# Autodesk Inventor assembly: Mini Power Module (REV-11-1956)
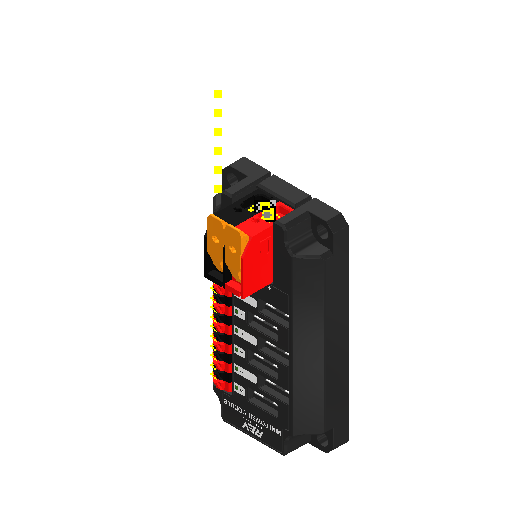
[picture p0: Inventor's stored thumbnail of the model, 512x512]
Saved by Autodesk Inventor 2023 (Build 270158000, 158)
## iProperties
Created: 2023-04-23
Part Number: Mini Power Module (REV-11-1956)
Description: STEP AP242
Document SubType Name: Assembly
Designer: adamarnold
Preprocessor: ST-DEVELOPER v18.102
Title: 64447f9ab2ee3a2914539952
## Documents named in this file (91)
- J:\My Drive\1939\2_Design\2023-2024\Parts\Electronics\Power Delivery\Mini Power Module (REV-11-1956).iam
- J:\My Drive\1939\2_Design\2023-2024\Parts\Electronics\MPM Parts\REV-11-1956.ipt
- J:\My Drive\1939\2_Design\2023-2024\Parts\Electronics\MPM Parts\REV-11-1956_1.ipt
- J:\My Drive\1939\2_Design\2023-2024\Parts\Electronics\MPM Parts\REV-11-1956_2.ipt
- J:\My Drive\1939\2_Design\2023-2024\Parts\Electronics\MPM Parts\REV-11-1956_3.ipt
- J:\My Drive\1939\2_Design\2023-2024\Parts\Electronics\MPM Parts\REV-11-1956_4.ipt
- J:\My Drive\1939\2_Design\2023-2024\Parts\Electronics\MPM Parts\REV-11-1956_5.ipt
- J:\My Drive\1939\2_Design\2023-2024\Parts\Electronics\MPM Parts\REV-11-1956_7.ipt
- J:\My Drive\1939\2_Design\2023-2024\Parts\Electronics\MPM Parts\REV-11-1956_8.ipt
- J:\My Drive\1939\2_Design\2023-2024\Parts\Electronics\MPM Parts\REV-11-1956_9.ipt
- J:\My Drive\1939\2_Design\2023-2024\Parts\Electronics\MPM Parts\REV-11-1956_10.ipt
- J:\My Drive\1939\2_Design\2023-2024\Parts\Electronics\MPM Parts\REV-11-1956_11.ipt
- J:\My Drive\1939\2_Design\2023-2024\Parts\Electronics\MPM Parts\REV-11-1956_12.ipt
- J:\My Drive\1939\2_Design\2023-2024\Parts\Electronics\MPM Parts\REV-11-1956_14.ipt
- J:\My Drive\1939\2_Design\2023-2024\Parts\Electronics\MPM Parts\REV-11-1956_15.ipt
- J:\My Drive\1939\2_Design\2023-2024\Parts\Electronics\MPM Parts\REV-11-1956_16.ipt
- J:\My Drive\1939\2_Design\2023-2024\Parts\Electronics\MPM Parts\REV-11-1956_17.ipt
- J:\My Drive\1939\2_Design\2023-2024\Parts\Electronics\MPM Parts\REV-11-1956_18.ipt
- J:\My Drive\1939\2_Design\2023-2024\Parts\Electronics\MPM Parts\REV-11-1956_19.ipt
- J:\My Drive\1939\2_Design\2023-2024\Parts\Electronics\MPM Parts\REV-11-1956_20.ipt
- J:\My Drive\1939\2_Design\2023-2024\Parts\Electronics\MPM Parts\REV-11-1956_22.ipt
- J:\My Drive\1939\2_Design\2023-2024\Parts\Electronics\MPM Parts\REV-11-1956_23.ipt
- J:\My Drive\1939\2_Design\2023-2024\Parts\Electronics\MPM Parts\REV-11-1956_24.ipt
- J:\My Drive\1939\2_Design\2023-2024\Parts\Electronics\MPM Parts\REV-11-1956_25.ipt
- J:\My Drive\1939\2_Design\2023-2024\Parts\Electronics\MPM Parts\REV-11-1956_26.ipt
- J:\My Drive\1939\2_Design\2023-2024\Parts\Electronics\MPM Parts\REV-11-1956_27.ipt
- J:\My Drive\1939\2_Design\2023-2024\Parts\Electronics\MPM Parts\REV-11-1956_29.ipt
- J:\My Drive\1939\2_Design\2023-2024\Parts\Electronics\MPM Parts\REV-11-1956_30.ipt
- J:\My Drive\1939\2_Design\2023-2024\Parts\Electronics\MPM Parts\REV-11-1956_31.ipt
- J:\My Drive\1939\2_Design\2023-2024\Parts\Electronics\MPM Parts\REV-11-1956_32.ipt
- J:\My Drive\1939\2_Design\2023-2024\Parts\Electronics\MPM Parts\REV-11-1956_33.ipt
- J:\My Drive\1939\2_Design\2023-2024\Parts\Electronics\MPM Parts\REV-11-1956_34.ipt
- J:\My Drive\1939\2_Design\2023-2024\Parts\Electronics\MPM Parts\REV-11-1956_35.ipt
- J:\My Drive\1939\2_Design\2023-2024\Parts\Electronics\MPM Parts\REV-11-1956_36.ipt
- J:\My Drive\1939\2_Design\2023-2024\Parts\Electronics\MPM Parts\REV-11-1956_37.ipt
- J:\My Drive\1939\2_Design\2023-2024\Parts\Electronics\MPM Parts\REV-11-1956_38.ipt
- J:\My Drive\1939\2_Design\2023-2024\Parts\Electronics\MPM Parts\REV-11-1956_39.ipt
- J:\My Drive\1939\2_Design\2023-2024\Parts\Electronics\MPM Parts\REV-11-1956_40.ipt
- J:\My Drive\1939\2_Design\2023-2024\Parts\Electronics\MPM Parts\REV-11-1956_41.ipt
- J:\My Drive\1939\2_Design\2023-2024\Parts\Electronics\MPM Parts\REV-11-1956_42.ipt
- J:\My Drive\1939\2_Design\2023-2024\Parts\Electronics\MPM Parts\REV-11-1956_43.ipt
- J:\My Drive\1939\2_Design\2023-2024\Parts\Electronics\MPM Parts\REV-11-1956_46.ipt
- J:\My Drive\1939\2_Design\2023-2024\Parts\Electronics\MPM Parts\REV-11-1956_47.ipt
- J:\My Drive\1939\2_Design\2023-2024\Parts\Electronics\MPM Parts\REV-11-1956_48.ipt
- J:\My Drive\1939\2_Design\2023-2024\Parts\Electronics\MPM Parts\REV-11-1956_49.ipt
- J:\My Drive\1939\2_Design\2023-2024\Parts\Electronics\MPM Parts\REV-11-1956_50.ipt
- J:\My Drive\1939\2_Design\2023-2024\Parts\Electronics\MPM Parts\REV-11-1956_51.ipt
- J:\My Drive\1939\2_Design\2023-2024\Parts\Electronics\MPM Parts\REV-11-1956_52.ipt
- J:\My Drive\1939\2_Design\2023-2024\Parts\Electronics\MPM Parts\REV-11-1956_53.ipt
- J:\My Drive\1939\2_Design\2023-2024\Parts\Electronics\MPM Parts\REV-11-1956_54.ipt
- J:\My Drive\1939\2_Design\2023-2024\Parts\Electronics\MPM Parts\REV-11-1956_55.ipt
- J:\My Drive\1939\2_Design\2023-2024\Parts\Electronics\MPM Parts\REV-11-1956_57.ipt
- J:\My Drive\1939\2_Design\2023-2024\Parts\Electronics\MPM Parts\REV-11-1956_58.ipt
- J:\My Drive\1939\2_Design\2023-2024\Parts\Electronics\MPM Parts\REV-11-1956_59.ipt
- J:\My Drive\1939\2_Design\2023-2024\Parts\Electronics\MPM Parts\REV-11-1956_60.ipt
- J:\My Drive\1939\2_Design\2023-2024\Parts\Electronics\MPM Parts\REV-11-1956_61.ipt
- J:\My Drive\1939\2_Design\2023-2024\Parts\Electronics\MPM Parts\REV-11-1956_63.ipt
- J:\My Drive\1939\2_Design\2023-2024\Parts\Electronics\MPM Parts\REV-11-1956_64.ipt
- J:\My Drive\1939\2_Design\2023-2024\Parts\Electronics\MPM Parts\REV-11-1956_65.ipt
- J:\My Drive\1939\2_Design\2023-2024\Parts\Electronics\MPM Parts\REV-11-1956_66.ipt
- J:\My Drive\1939\2_Design\2023-2024\Parts\Electronics\MPM Parts\REV-11-1956_67.ipt
- J:\My Drive\1939\2_Design\2023-2024\Parts\Electronics\MPM Parts\REV-11-1956_68.ipt
- J:\My Drive\1939\2_Design\2023-2024\Parts\Electronics\MPM Parts\REV-11-1956_69.ipt
- J:\My Drive\1939\2_Design\2023-2024\Parts\Electronics\MPM Parts\REV-11-1956_71.ipt
- J:\My Drive\1939\2_Design\2023-2024\Parts\Electronics\MPM Parts\REV-11-1956_72.ipt
- J:\My Drive\1939\2_Design\2023-2024\Parts\Electronics\MPM Parts\REV-11-1956_73.ipt
- J:\My Drive\1939\2_Design\2023-2024\Parts\Electronics\MPM Parts\REV-11-1956_74.ipt
- J:\My Drive\1939\2_Design\2023-2024\Parts\Electronics\MPM Parts\REV-11-1956_75.ipt
- J:\My Drive\1939\2_Design\2023-2024\Parts\Electronics\MPM Parts\REV-11-1956_76.ipt
- J:\My Drive\1939\2_Design\2023-2024\Parts\Electronics\MPM Parts\REV-11-1956_77.ipt
- J:\My Drive\1939\2_Design\2023-2024\Parts\Electronics\MPM Parts\REV-11-1956_78.ipt
- J:\My Drive\1939\2_Design\2023-2024\Parts\Electronics\MPM Parts\REV-11-1956_79.ipt
- J:\My Drive\1939\2_Design\2023-2024\Parts\Electronics\MPM Parts\REV-11-1956_80.ipt
- J:\My Drive\1939\2_Design\2023-2024\Parts\Electronics\MPM Parts\REV-11-1956_81.ipt
- J:\My Drive\1939\2_Design\2023-2024\Parts\Electronics\MPM Parts\REV-11-1956_82.ipt
- J:\My Drive\1939\2_Design\2023-2024\Parts\Electronics\MPM Parts\REV-11-1956_85.ipt
- J:\My Drive\1939\2_Design\2023-2024\Parts\Electronics\MPM Parts\REV-11-1956_86.ipt
- J:\My Drive\1939\2_Design\2023-2024\Parts\Electronics\MPM Parts\REV-11-1956_87.ipt
- J:\My Drive\1939\2_Design\2023-2024\Parts\Electronics\MPM Parts\REV-11-1956_88.ipt
- J:\My Drive\1939\2_Design\2023-2024\Parts\Electronics\MPM Parts\REV-11-1956_89.ipt
- J:\My Drive\1939\2_Design\2023-2024\Parts\Electronics\MPM Parts\REV-11-1956_90.ipt
- J:\My Drive\1939\2_Design\2023-2024\Parts\Electronics\MPM Parts\REV-11-1956_91.ipt
- J:\My Drive\1939\2_Design\2023-2024\Parts\Electronics\MPM Parts\REV-11-1956_92.ipt
- J:\My Drive\1939\2_Design\2023-2024\Parts\Electronics\MPM Parts\REV-11-1956_93.ipt
- J:\My Drive\1939\2_Design\2023-2024\Parts\Electronics\MPM Parts\REV-11-1956_94.ipt
- J:\My Drive\1939\2_Design\2023-2024\Parts\Electronics\MPM Parts\REV-11-1956_95.ipt
- J:\My Drive\1939\2_Design\2023-2024\Parts\Electronics\MPM Parts\REV-11-1956_96.ipt
- J:\My Drive\1939\2_Design\2023-2024\Parts\Electronics\MPM Parts\REV-11-1956_98.ipt
- J:\My Drive\1939\2_Design\2023-2024\Parts\Electronics\MPM Parts\REV-11-1956_99.ipt
- J:\My Drive\1939\2_Design\2023-2024\Parts\Electronics\PDH Parts\Positive_small.ipt
- J:\My Drive\1939\2_Design\2023-2024\Parts\Electronics\PDH Parts\Negative_small.ipt
## Components (100 placed, 90 different names)
1. NAUO1
2. NAUO2
3. NAUO3
4. NAUO4
5. NAUO5
6. NAUO6
7. NAUO8
8. NAUO9
9. NAUO10
10. NAUO11
11. NAUO12
12. NAUO13
13. NAUO15
14. NAUO16
15. NAUO17
16. NAUO18
17. NAUO19
18. NAUO20
19. NAUO21
20. NAUO23
21. NAUO24
22. NAUO25
23. NAUO26
24. NAUO27
25. NAUO28
26. NAUO30
27. NAUO31
28. NAUO32
29. NAUO33
30. NAUO34
31. NAUO35
32. NAUO36
33. NAUO37
34. NAUO38
35. NAUO39
36. NAUO40
37. NAUO41
38. NAUO42
39. NAUO43
40. NAUO44
41. NAUO47
42. NAUO48
43. NAUO49
44. NAUO50
45. NAUO51
46. NAUO52
47. NAUO53
48. NAUO54
49. NAUO55
50. NAUO56
51. NAUO58
52. NAUO59
53. NAUO60
54. NAUO61
55. NAUO62
56. NAUO64
57. NAUO65
58. NAUO66
59. NAUO67
60. NAUO68
61. NAUO69
62. NAUO70
63. NAUO72
64. NAUO73
65. NAUO74
66. NAUO75
67. NAUO76
68. NAUO77
69. NAUO78
70. NAUO79
71. NAUO80
72. NAUO81 — Mate:1, Flush:1, Flush:2, Mate:2
73. NAUO82
74. NAUO83
75. NAUO86
76. NAUO87
77. NAUO88
78. NAUO89
79. NAUO90
80. NAUO91
81. NAUO92
82. NAUO93
83. NAUO94
84. NAUO95
85. NAUO96
86. NAUO97
87. NAUO99
88. NAUO100
89. Positive_small:1 — Mate:1, Flush:1, Flush:2, Flush:3, Mate:3, Flush:14, Flush:22, Flush:23
90. Negative_small:1 — Flush:3, Mate:2, Mate:3, Flush:15, Mate:9
91. Positive_small:2 — Flush:5, Flush:14, Flush:15, Mate:9
92. Negative_small:2 — Flush:5, Flush:8, Flush:9, Mate:6
93. Positive_small:3 — Flush:8, Flush:9, Mate:6
94. Negative_small:3 — Flush:12, Mate:8, Flush:13
95. Positive_small:4 — Flush:12, Mate:8, Flush:13
96. Negative_small:4 — Mate:13
97. Positive_small:5 — Flush:20, Flush:21, Mate:12, Flush:22, Flush:23
98. Negative_small:5
99. Positive_small:6 — Flush:20, Flush:21, Mate:13
100. Negative_small:6 — Mate:12
## Relationships (36: Flush 23, Mate 13)
- Mate:1: NAUO81 ↔ Positive_small:1
- Flush:1 (10.0584 mm): NAUO81 ↔ Positive_small:1
- Flush:2: NAUO81 ↔ Positive_small:1
- Flush:3: Positive_small:1 ↔ Negative_small:1
- Mate:2: NAUO81 ↔ Negative_small:1
- Mate:3: Positive_small:1 ↔ Negative_small:1
- [Flush]: Positive_small:2 ↔ Negative_small:2
- [Mate]: Positive_small:2 ↔ Negative_small:2
- Flush:5: Positive_small:2 ↔ Negative_small:2
- [Flush]: Positive_small:3 ↔ Negative_small:3
- [Mate]: Positive_small:3 ↔ Negative_small:3
- [Flush]: Positive_small:3 ↔ Negative_small:3
- Flush:8: Negative_small:2 ↔ Positive_small:3
- Flush:9: Negative_small:2 ↔ Positive_small:3
- Mate:6: Negative_small:2 ↔ Positive_small:3
- [Flush]: Positive_small:4 ↔ Negative_small:4
- [Mate]: Positive_small:4 ↔ Negative_small:4
- [Flush]: Positive_small:4 ↔ Negative_small:4
- Flush:12: Negative_small:3 ↔ Positive_small:4
- Mate:8: Negative_small:3 ↔ Positive_small:4
- Flush:13: Negative_small:3 ↔ Positive_small:4
- Flush:14: Positive_small:1 ↔ Positive_small:2
- Flush:15: Negative_small:1 ↔ Positive_small:2
- Mate:9: Negative_small:1 ↔ Positive_small:2
- [Flush]: Positive_small:5 ↔ Negative_small:5
- [Mate]: Positive_small:5 ↔ Negative_small:5
- [Flush]: Positive_small:5 ↔ Negative_small:5
- [Flush]: Positive_small:6 ↔ Negative_small:6
- [Mate]: Positive_small:6 ↔ Negative_small:6
- [Flush]: Positive_small:6 ↔ Negative_small:6
- Flush:20: Positive_small:5 ↔ Positive_small:6
- Flush:21: Positive_small:5 ↔ Positive_small:6
- Mate:12: Positive_small:5 ↔ Negative_small:6
- Flush:22: Positive_small:1 ↔ Positive_small:5
- Flush:23: Positive_small:1 ↔ Positive_small:5
- Mate:13: Negative_small:4 ↔ Positive_small:6
## Named parameters: d6_d3 = 0 mm, d7_d5 = 0 mm, d9_d6_d3 = 0 mm, d10_d7_d5 = 0 mm, d11_d8 = 0 mm, d15_d6_d3 = 0 mm, d16_d7_d5 = 0 mm, d17_d8 = 0 mm, d24_d15_d6_d3 = 0 mm, d25_d16_d7_d5 = 0 mm, d26_d17_d8 = 0 mm, d27_d15_d6_d3 = 0 mm, d28_d16_d7_d5 = 0 mm, d29_d17_d8 = 0 mm
